# Autodesk Inventor assembly: Assembly_spindeldrive_350mm
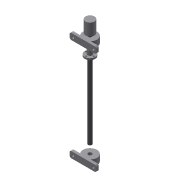
[picture p0: Inventor's stored thumbnail of the model, 180x180]
Saved by Autodesk Inventor 2019.4 (Build 234330000, 330)
## iProperties
Created: 2020-10-27
Part Number: Assembly_spindeldrive_350mm
Document SubType Name: Assembly
Designer: diederichbenedict
Author: diederichbenedict
## Documents named in this file (4)
- C:\Users\diederichbenedict\Dropbox\Dokumente\Promotion\PROJECTS\OPENTRONS\INVENTOR\Assembly_spindeldrive_350mm_2.iam
- C:\Users\diederichbenedict\Dropbox\Dokumente\Promotion\PROJECTS\OPENTRONS\INVENTOR\00_spindel_350mm.ipt
- C:\Users\diederichbenedict\Dropbox\Dokumente\Promotion\PROJECTS\OPENTRONS\INVENTOR\00_spindel_bearings.ipt
- C:\Users\diederichbenedict\Dropbox\Dokumente\Promotion\PROJECTS\OPENTRONS\INVENTOR\00_spindel_slide.ipt
## Components (4 placed, 3 different names)
1. 00_spindel_350mm:1 — Mate:1, Mate:2, Mate:3, Mate:6
2. 00_spindel_bearings:1 — Mate:2, Angle:2, Mate:5
3. 00_spindel_bearings:2 — Mate:1, Angle:1, Angle:2, Angle:3, Mate:5, Mate:6, Mate:4
4. 00_spindel_slide:1 — Mate:3, Angle:3, Mate:4
## Relationships (9: Mate 6, Angle 3)
- Mate:1: 00_spindel_350mm:1 ↔ 00_spindel_bearings:2
- Mate:2: 00_spindel_350mm:1 ↔ 00_spindel_bearings:1
- Angle:1 (180 deg): 00_spindel_bearings:2
- Angle:2 (0 deg): 00_spindel_bearings:1 ↔ 00_spindel_bearings:2
- Mate:3: 00_spindel_350mm:1 ↔ 00_spindel_slide:1
- Angle:3 (0 deg): 00_spindel_bearings:2 ↔ 00_spindel_slide:1
- Mate:4 (20 mm): 00_spindel_bearings:2 ↔ 00_spindel_slide:1
- Mate:5 (200 mm): 00_spindel_bearings:1 ↔ 00_spindel_bearings:2
- Mate:6 (5 mm): 00_spindel_350mm:1 ↔ 00_spindel_bearings:2
